# Autodesk Inventor assembly: CONTROLBOARDAS
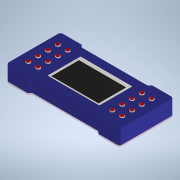
[picture p0: Inventor's stored thumbnail of the model, 180x180]
Saved by Autodesk Inventor 2020 (Build 240168000, 168)
## iProperties
Created: 2020-06-05
Part Number: CONTROLBOARDAS
Document SubType Name: Assembly
Designer: Gebruiker
Author: Gebruiker
## Documents named in this file (12)
- C:\Users\Gebruiker\Documents\GitHub\BeerMinder\3D-model\ControlBox\CONTROLBOARDAS.iam
- C:\Users\Gebruiker\Documents\GitHub\BeerMinder\3D-model\ControlBox\CONTROL_BOARD.ipt
- C:\Users\Gebruiker\Documents\GitHub\BeerMinder\3D-model\ControlBox\Nextion 4.3 Enhanced v10.ipt
- C:\Users\Gebruiker\Documents\GitHub\BeerMinder\3D-model\ControlBox\Tactal Switch - THRU(12mmx12mm - Illuminated - Red.ipt
- C:\Users\Gebruiker\Documents\GitHub\BeerMinder\3D-model\ControlBox\ScrewTerminal\ScrewTerminal.iam
- C:\Users\Gebruiker\Documents\GitHub\BeerMinder\3D-model\controller\PCB2_MIR.ipt
- C:\Users\Gebruiker\Documents\GitHub\BeerMinder\3D-model\controller\CONTROLBOARD_KLEP.ipt
- C:\Users\Gebruiker\Documents\GitHub\BeerMinder\3D-model\controller\KLEP_KNOPPEN.ipt
- C:\Users\Gebruiker\Documents\GitHub\BeerMinder\3D-model\controller\KLEP_KNOPPEN_MIR.ipt
- C:\Users\Gebruiker\Documents\GitHub\BeerMinder\3D-model\controller\PCB2_MIR_MIR2.ipt
- C:\Users\Gebruiker\Documents\GitHub\BeerMinder\3D-model\ControlBox\Tactal Switch - THRU(12mmx12mm - Illuminated - Red_MIR.ipt
- C:\Users\Gebruiker\Documents\GitHub\BeerMinder\3D-model\controller\KLEPKNOP2.ipt
## Components (57 placed, 11 different names)
1. CONTROL_BOARD:1 — Mate:1, Angle:1, Angle:2, Mate:4, Mate:5, Flush:1, Angle:16, Mate:18, Angle:19, Mate:21, Mate:22, Mate:24, Mate:26, Flush:22, Flush:23
2. Nextion 4.3 Enhanced v10:1 — Mate:1, Angle:1, Angle:2, Angle:16, Mate:21, Mate:22, Flush:12, Flush:13, Flush:16, Flush:17
3. PCB2_MIR:1 — Mate:23, Flush:10, Flush:11, Mate:24, Flush:12, Flush:13, Mate:27, Angle:21, Mate:28, Mate:29, Angle:22, Mate:30
4. CONTROLBOARD_KLEP:1 — Mate:18, Angle:19, Mate:20, Angle:20, Mate:35, Flush:18, Flush:19, Mate:36, Flush:20, Flush:21, Flush:22, Flush:23, Mate:37, Flush:24, Mate:38, Flush:25
5. KLEP_KNOPPEN:2 — Mate:20, Angle:20, Mate:38, Flush:25
6. KLEP_KNOPPEN_MIR:1 — Mate:37, Flush:24
7. PCB2_MIR_MIR2:1 — Flush:14, Flush:15, Mate:25, Flush:16, Flush:17, Mate:26, Mate:31, Angle:23, Mate:32, Mate:33, Angle:24, Mate:34
8. KLEPKNOP2:1 — Mate:35, Flush:18, Flush:19
9. KLEPKNOP2:2 — Mate:36, Flush:20, Flush:21
10. Tactal Switch - THRU(12mmx12mm - Illuminated - Red:5
11. Tactal Switch - THRU(12mmx12mm - Illuminated - Red:8
12. Tactal Switch - THRU(12mmx12mm - Illuminated - Red:9
13. Tactal Switch - THRU(12mmx12mm - Illuminated - Red:10
14. Tactal Switch - THRU(12mmx12mm - Illuminated - Red:11
15. Tactal Switch - THRU(12mmx12mm - Illuminated - Red:12
16. Tactal Switch - THRU(12mmx12mm - Illuminated - Red:13
17. Tactal Switch - THRU(12mmx12mm - Illuminated - Red:14
18. Tactal Switch - THRU(12mmx12mm - Illuminated - Red:1 — Mate:23, Flush:10, Flush:11
19. Tactal Switch - THRU(12mmx12mm - Illuminated - Red:22
20. Tactal Switch - THRU(12mmx12mm - Illuminated - Red:23
21. Tactal Switch - THRU(12mmx12mm - Illuminated - Red:24
22. Tactal Switch - THRU(12mmx12mm - Illuminated - Red:25
23. Tactal Switch - THRU(12mmx12mm - Illuminated - Red:26
24. Tactal Switch - THRU(12mmx12mm - Illuminated - Red:27
25. Tactal Switch - THRU(12mmx12mm - Illuminated - Red:28
26. Tactal Switch - THRU(12mmx12mm - Illuminated - Red_MIR:1 — Flush:14, Flush:15, Mate:25
27. Tactal Switch - THRU(12mmx12mm - Illuminated - Red_MIR:2
28. Tactal Switch - THRU(12mmx12mm - Illuminated - Red_MIR:3
29. Tactal Switch - THRU(12mmx12mm - Illuminated - Red_MIR:4
30. Tactal Switch - THRU(12mmx12mm - Illuminated - Red_MIR:5
31. Tactal Switch - THRU(12mmx12mm - Illuminated - Red_MIR:6
32. Tactal Switch - THRU(12mmx12mm - Illuminated - Red_MIR:7
33. Tactal Switch - THRU(12mmx12mm - Illuminated - Red_MIR:8
34. ScrewTerminal:2 [sub-assembly] — Mate:27, Angle:21, Mate:28
35. ScrewTerminal:4 [sub-assembly]
36. ScrewTerminal:5 [sub-assembly]
37. ScrewTerminal:6 [sub-assembly]
38. ScrewTerminal:7 [sub-assembly]
39. ScrewTerminal:8 [sub-assembly]
40. ScrewTerminal:3 [sub-assembly] — Mate:29, Angle:22, Mate:30
41. ScrewTerminal:9 [sub-assembly]
42. ScrewTerminal:10 [sub-assembly]
43. ScrewTerminal:11 [sub-assembly]
44. ScrewTerminal:12 [sub-assembly]
45. ScrewTerminal:13 [sub-assembly]
46. ScrewTerminal:15 [sub-assembly] — Mate:33, Angle:24, Mate:34
47. ScrewTerminal:16 [sub-assembly]
48. ScrewTerminal:17 [sub-assembly]
49. ScrewTerminal:18 [sub-assembly]
50. ScrewTerminal:19 [sub-assembly]
51. ScrewTerminal:20 [sub-assembly]
52. ScrewTerminal:14 [sub-assembly] — Mate:31, Angle:23, Mate:32
53. ScrewTerminal:21 [sub-assembly]
54. ScrewTerminal:22 [sub-assembly]
55. ScrewTerminal:23 [sub-assembly]
56. ScrewTerminal:24 [sub-assembly]
57. ScrewTerminal:25 [sub-assembly]
## Component patterns: (8 elements, first: Tactal Switch - THRU(12mmx12mm - Illuminated - Red:5), (8 elements, first: Tactal Switch - THRU(12mmx12mm - Illuminated - Red:1), (8 elements, first: Tactal Switch - THRU(12mmx12mm - Illuminated - Red_MIR:1), (6 elements, first: ScrewTerminal:2), (6 elements, first: ScrewTerminal:3), (6 elements, first: ScrewTerminal:15), (6 elements, first: ScrewTerminal:14)
## Relationships (49: Mate 23, Flush 17, Angle 9)
- Mate:1: CONTROL_BOARD:1 ↔ Nextion 4.3 Enhanced v10:1
- Angle:1 (0 deg): CONTROL_BOARD:1 ↔ Nextion 4.3 Enhanced v10:1
- Angle:2 (0 deg): CONTROL_BOARD:1 ↔ Nextion 4.3 Enhanced v10:1
- Mate:4: CONTROL_BOARD:1
- Mate:5: CONTROL_BOARD:1
- Flush:1: CONTROL_BOARD:1
- Angle:16 (0 deg): CONTROL_BOARD:1 ↔ Nextion 4.3 Enhanced v10:1
- Mate:18: CONTROL_BOARD:1 ↔ CONTROLBOARD_KLEP:1
- Angle:19 (0 deg): CONTROL_BOARD:1 ↔ CONTROLBOARD_KLEP:1
- Mate:20: CONTROLBOARD_KLEP:1 ↔ KLEP_KNOPPEN:2
- Angle:20 (0 deg): CONTROLBOARD_KLEP:1 ↔ KLEP_KNOPPEN:2
- Mate:21 (7 mm): CONTROL_BOARD:1 ↔ Nextion 4.3 Enhanced v10:1
- Mate:22 (49 mm): CONTROL_BOARD:1 ↔ Nextion 4.3 Enhanced v10:1
- Mate:23: PCB2_MIR:1 ↔ Tactal Switch - THRU(12mmx12mm - Illuminated - Red:1
- Flush:10 (7 mm): PCB2_MIR:1 ↔ Tactal Switch - THRU(12mmx12mm - Illuminated - Red:1
- Flush:11 (4.3 mm): PCB2_MIR:1 ↔ Tactal Switch - THRU(12mmx12mm - Illuminated - Red:1
- Mate:24: CONTROL_BOARD:1 ↔ PCB2_MIR:1
- Flush:12 (-5.2 mm): Nextion 4.3 Enhanced v10:1 ↔ PCB2_MIR:1
- Flush:13 (122.7 mm): Nextion 4.3 Enhanced v10:1 ↔ PCB2_MIR:1
- Flush:14 (4.3 mm): PCB2_MIR_MIR2:1 ↔ Tactal Switch - THRU(12mmx12mm - Illuminated - Red_MIR:1
- Flush:15 (7 mm): PCB2_MIR_MIR2:1 ↔ Tactal Switch - THRU(12mmx12mm - Illuminated - Red_MIR:1
- Mate:25: PCB2_MIR_MIR2:1 ↔ Tactal Switch - THRU(12mmx12mm - Illuminated - Red_MIR:1
- Flush:16 (122.7 mm): Nextion 4.3 Enhanced v10:1 ↔ PCB2_MIR_MIR2:1
- Flush:17 (-5.2 mm): Nextion 4.3 Enhanced v10:1 ↔ PCB2_MIR_MIR2:1
- Mate:26: CONTROL_BOARD:1 ↔ PCB2_MIR_MIR2:1
- Mate:27: PCB2_MIR:1 ↔ ScrewTerminal:2
- Angle:21 (0 deg): PCB2_MIR:1 ↔ ScrewTerminal:2
- Mate:28: PCB2_MIR:1 ↔ ScrewTerminal:2
- Mate:29: PCB2_MIR:1 ↔ ScrewTerminal:3
- Angle:22 (0 deg): PCB2_MIR:1 ↔ ScrewTerminal:3
- Mate:30: PCB2_MIR:1 ↔ ScrewTerminal:3
- Mate:31: PCB2_MIR_MIR2:1 ↔ ScrewTerminal:14
- Angle:23 (0 deg): PCB2_MIR_MIR2:1 ↔ ScrewTerminal:14
- Mate:32: PCB2_MIR_MIR2:1 ↔ ScrewTerminal:14
- Mate:33: PCB2_MIR_MIR2:1 ↔ ScrewTerminal:15
- Angle:24 (0 deg): PCB2_MIR_MIR2:1 ↔ ScrewTerminal:15
- Mate:34: PCB2_MIR_MIR2:1 ↔ ScrewTerminal:15
- Mate:35: CONTROLBOARD_KLEP:1 ↔ KLEPKNOP2:1
- Flush:18 (14 mm): CONTROLBOARD_KLEP:1 ↔ KLEPKNOP2:1
- Flush:19 (3 mm): CONTROLBOARD_KLEP:1 ↔ KLEPKNOP2:1
- Mate:36: CONTROLBOARD_KLEP:1 ↔ KLEPKNOP2:2
- Flush:20 (14 mm): CONTROLBOARD_KLEP:1 ↔ KLEPKNOP2:2
- Flush:21 (3 mm): CONTROLBOARD_KLEP:1 ↔ KLEPKNOP2:2
- Flush:22: CONTROL_BOARD:1 ↔ CONTROLBOARD_KLEP:1
- Flush:23: CONTROL_BOARD:1 ↔ CONTROLBOARD_KLEP:1
- Mate:37: CONTROLBOARD_KLEP:1 ↔ KLEP_KNOPPEN_MIR:1
- Flush:24 (19.5 mm): CONTROLBOARD_KLEP:1 ↔ KLEP_KNOPPEN_MIR:1
- Mate:38: CONTROLBOARD_KLEP:1 ↔ KLEP_KNOPPEN:2
- Flush:25 (19.5 mm): CONTROLBOARD_KLEP:1 ↔ KLEP_KNOPPEN:2
